# Autodesk Inventor assembly: montagem_teste
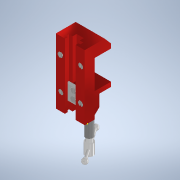
[picture p0: Inventor's stored thumbnail of the model, 180x180]
Saved by Autodesk Inventor 2022.2 (Build 262287010, 287A)
## iProperties
Created: 2022-03-09
Part Number: montagem_teste
Document SubType Name: Assembly
Designer: Korch
Author: Korch
## Documents named in this file (10)
- C:\Users\Usuario\Desktop\Faculdade\modelagem_3D\morsa\montagem_teste.iam
- C:\Users\Usuario\Desktop\Faculdade\modelagem_3D\morsa\morsa_body.ipt
- C:\Users\Usuario\Desktop\Faculdade\modelagem_3D\morsa\haste_roscada.ipt
- C:\Users\Usuario\Desktop\Faculdade\modelagem_3D\morsa\mordente_movel.ipt
- C:\Users\Usuario\Desktop\Faculdade\modelagem_3D\morsa\parafuso_de_trava.ipt
- C:\Users\Usuario\Desktop\Faculdade\modelagem_3D\morsa\grampo_trava.ipt
- C:\Users\Usuario\Desktop\Faculdade\modelagem_3D\morsa\chapa_base.ipt
- C:\Users\Usuario\Desktop\Faculdade\modelagem_3D\morsa\manipulo.ipt
- C:\Users\Usuario\Desktop\Faculdade\modelagem_3D\morsa\esfera.ipt
- C:\Users\Usuario\Documents\Inventor\Content Center Files\R2022\en-US\DIN 963\DIN 963 - M6 x 16.ipt
## Components (16 placed, 9 different names)
1. morsa_body:1 — Insert:4, Insert:5, Insert:6, Insert:7, Mate:1, Mate:2, Rotation/Translation:1, Cylindrical:1, Mate:10
2. haste_roscada:1 — Insert:1, Rotation/Translation:1, Rotation:1, Rigid:3, Cylindrical:1
3. mordente_movel:1 — Insert:1, Insert:2, Insert:3, Mate:1, Mate:2, Mate:3, Mate:10
4. parafuso_de_trava:1 — Mate:3
5. grampo_trava:1 — Insert:2, Insert:3, Mate:8, Mate:9
6. chapa_base:1 — Insert:4, Insert:5, Mate:4, Mate:6
7. chapa_base:2 — Insert:6, Insert:7, Mate:5, Mate:7
8. manipulo:1 — Rigid:1, Rigid:2, Rotation:1, Rigid:3
9. esfera:1 — Rigid:2
10. esfera:2 — Rigid:1
11. DIN 963 - replaced by DIN EN ISO 2009 M6 x 16:1 — Mate:4
12. DIN 963 - replaced by DIN EN ISO 2009 M6 x 16:2 — Mate:7
13. DIN 963 - replaced by DIN EN ISO 2009 M6 x 16:3 — Mate:6
14. DIN 963 - replaced by DIN EN ISO 2009 M6 x 16:4 — Mate:9
15. DIN 963 - replaced by DIN EN ISO 2009 M6 x 16:5 — Mate:5
16. DIN 963 - replaced by DIN EN ISO 2009 M6 x 16:6 — Mate:8
## Relationships (25: Mate 10, Insert 7, WeldJoint 3, Flush 2, RelateRotateTranslate 1, RelateRotation 1, CylindricalJoint 1)
- Insert:1: haste_roscada:1 ↔ mordente_movel:1
- Insert:2: mordente_movel:1 ↔ grampo_trava:1
- Insert:3: mordente_movel:1 ↔ grampo_trava:1
- Insert:4: morsa_body:1 ↔ chapa_base:1
- Insert:5: morsa_body:1 ↔ chapa_base:1
- Insert:6: morsa_body:1 ↔ chapa_base:2
- Insert:7: morsa_body:1 ↔ chapa_base:2
- Rigid:1 [WeldJoint]: manipulo:1 ↔ esfera:2
- Rigid:2 [WeldJoint]: manipulo:1 ↔ esfera:1
- Mate:1 (10 mm): morsa_body:1 ↔ mordente_movel:1
- Mate:2: morsa_body:1 ↔ mordente_movel:1
- Mate:3: mordente_movel:1 ↔ parafuso_de_trava:1
- Mate:4: chapa_base:1 ↔ DIN 963 - replaced by DIN EN ISO 2009 M6 x 16:1
- Mate:5: chapa_base:2 ↔ DIN 963 - replaced by DIN EN ISO 2009 M6 x 16:5
- Mate:6: chapa_base:1 ↔ DIN 963 - replaced by DIN EN ISO 2009 M6 x 16:3
- Mate:7: chapa_base:2 ↔ DIN 963 - replaced by DIN EN ISO 2009 M6 x 16:2
- Mate:8: grampo_trava:1 ↔ DIN 963 - replaced by DIN EN ISO 2009 M6 x 16:6
- Mate:9: grampo_trava:1 ↔ DIN 963 - replaced by DIN EN ISO 2009 M6 x 16:4
- Rotation/Translation:1 [RelateRotateTranslate] (50.265 mm): morsa_body:1 ↔ haste_roscada:1
- Rotation:1 [RelateRotation] (1 ul): haste_roscada:1 ↔ manipulo:1
- Rigid:3 [WeldJoint]: haste_roscada:1 ↔ manipulo:1
- Cylindrical:1: morsa_body:1 ↔ haste_roscada:1
- Flush:1 (-44.009 mm)
- Flush:2 (41.991 mm)
- Mate:10: morsa_body:1 ↔ mordente_movel:1
